# Autodesk Inventor assembly: 42146-28
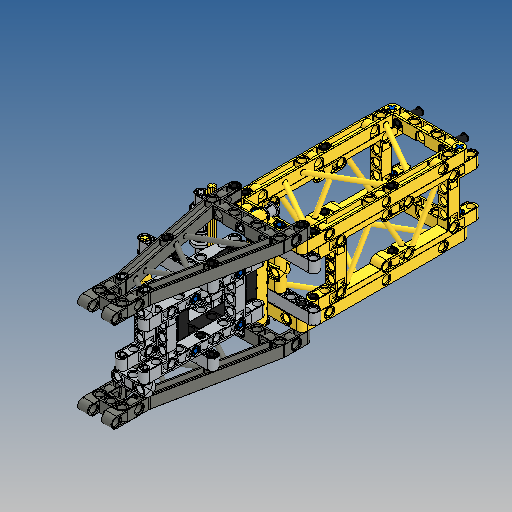
[picture p0: Inventor's stored thumbnail of the model, 512x512]
Saved by Autodesk Inventor 2025 (Build 290162010, 162A)
## iProperties
Created: 2024-12-04
Part Number: 42146-28
Material: Generisch
Document SubType Name: Assembly
Designer: hp.muther
Author: hp.muther
## Documents named in this file (22)
- D:\Inventor\Projekte\Muther\LEGO Technic\LEGO Technik - Raupenkran LR 13000 (42146)\42146-28.iam
- D:\Inventor\Projekte\Muther\LEGO Technic\LEGO Pieces\Rahmen, T-Stücke\79766-Yellow.ipt
- D:\Inventor\Projekte\Muther\LEGO Technic\LEGO Pieces\Pin's\2780-Black.ipt
- D:\Inventor\Projekte\Muther\LEGO Technic\LEGO Pieces\Pin's\43093-Blue.ipt
- D:\Inventor\Projekte\Muther\LEGO Technic\LEGO Pieces\Rahmen, T-Stücke\79767-Yellow.ipt
- D:\Inventor\Projekte\Muther\LEGO Technic\LEGO Pieces\Verbindungselemente\39793-Yellow.ipt
- D:\Inventor\Projekte\Muther\LEGO Technic\LEGO Pieces\Pin's\6558-Blue.ipt
- D:\Inventor\Projekte\Muther\LEGO Technic\LEGO Pieces\Lochbalken\32525-LtBluishGray.ipt
- D:\Inventor\Projekte\Muther\LEGO Technic\LEGO Pieces\Räder, Raupe\42610-LtBluishGray.ipt
- D:\Inventor\Projekte\Muther\LEGO Technic\LEGO Pieces\Rund\3713-LtBluishGray.ipt
- D:\Inventor\Projekte\Muther\LEGO Technic\LEGO Pieces\Rund\4265c-Yellow.ipt
- D:\Inventor\Projekte\Muther\LEGO Technic\LEGO Pieces\Achsen\32073-LtBluishGray.ipt
- D:\Inventor\Projekte\Muther\LEGO Technic\LEGO Pieces\Achsen\44294-Yellow.ipt
- D:\Inventor\Projekte\Muther\LEGO Technic\LEGO Pieces\Lochbalken\40490-Yellow.ipt
- D:\Inventor\Projekte\Muther\LEGO Technic\LEGO Pieces\Rahmen, T-Stücke\64178-LtBluishGray.ipt
- D:\Inventor\Projekte\Muther\LEGO Technic\LEGO Pieces\Rahmen, T-Stücke\64179-Black.ipt
- D:\Inventor\Projekte\Muther\LEGO Technic\LEGO Pieces\Verbindungselemente\48989-LtBluishGray.ipt
- D:\Inventor\Projekte\Muther\LEGO Technic\LEGO Pieces\Lochbalken\32524-LtBluishGray.ipt
- D:\Inventor\Projekte\Muther\LEGO Technic\LEGO Pieces\Rund\62462-Yellow.ipt
- D:\Inventor\Projekte\Muther\LEGO Technic\LEGO Pieces\Rahmen, T-Stücke\79768-DkBluishGray.ipt
- D:\Inventor\Projekte\Muther\LEGO Technic\LEGO Pieces\Pin's\18651-Black.ipt
- D:\Inventor\Projekte\Muther\LEGO Technic\LEGO Pieces\Pin's\32054-LtBluishGray.ipt
## Components (72 placed, 21 different names)
1. 79766-Yellow:1 — Einfügen:71, Einfügen:70, Einfügen:24, Einfügen:25, Einfügen:27, Einfügen:28, Einfügen:30, Einfügen:29, Einfügen:61, Einfügen:62, Einfügen:31, Einfügen:26, Einfügen:64
2. 2780-Black:1 — Einfügen:4
3. 2780-Black:2 — Einfügen:3
4. 2780-Black:3 — Einfügen:5
5. 2780-Black:4 — Einfügen:6
6. 2780-Black:5 — Einfügen:7
7. 43093-Blue:1 — Einfügen:2, Passend:2
8. 43093-Blue:2 — Einfügen:1, Passend:1
9. 79767-Yellow:1 — Einfügen:9, Passend:1
10. 79767-Yellow:2 — Einfügen:8, Passend:2, Einfügen:31, Passend:8
11. 39793-Yellow:1 — Einfügen:10, Einfügen:11, Einfügen:12, Einfügen:13, Einfügen:18, Einfügen:19
12. 6558-Blue:1 — Einfügen:10, Passend:7
13. 6558-Blue:2 — Einfügen:13
14. 6558-Blue:3 — Einfügen:11, Passend:3
15. 6558-Blue:4 — Einfügen:12
16. 32525-LtBluishGray:1 — Einfügen:19, Passend:4
17. 32525-LtBluishGray:2 — Einfügen:17, Einfügen:18, Passend:3, Einfügen:22, Einfügen:23
18. 42610-LtBluishGray:1 — Einfügen:16
19. 42610-LtBluishGray:2 — Einfügen:15, Einfügen:17
20. 3713-LtBluishGray:1 — Einfügen:14, Einfügen:15, Einfügen:16
21. 4265c-Yellow:1 — Einfügen:21, Passend:5
22. 4265c-Yellow:2 — Einfügen:20, Passend:6
23. 32073-LtBluishGray:1 — Einfügen:14, Passend:4
24. 44294-Yellow:1 — Einfügen:20, Einfügen:21, Passend:5, Passend:6, Einfügen:22
25. 79766-Yellow:2 — Einfügen:1, Einfügen:2, Einfügen:4, Einfügen:5, Einfügen:3, Einfügen:6, Einfügen:7, Einfügen:60, Einfügen:63, Einfügen:68, Einfügen:69, Passend:7, Einfügen:9, Einfügen:23, Einfügen:34, Einfügen:65, Einfügen:8
26. 2780-Black:6 — Einfügen:27
27. 2780-Black:7 — Einfügen:26, Passend:9
28. 2780-Black:8 — Einfügen:28
29. 2780-Black:9 — Einfügen:29
30. 2780-Black:10 — Einfügen:30
31. 43093-Blue:3 — Einfügen:25
32. 43093-Blue:4 — Einfügen:24, Passend:8
33. 6558-Blue:5 — Einfügen:32, Passend:18
34. 6558-Blue:6 — Einfügen:33
35. 40490-Yellow:1 — Einfügen:32, Einfügen:33, Einfügen:34, Passend:9, Einfügen:59, Einfügen:66, Einfügen:67
36. 64178-LtBluishGray:1 — Einfügen:40, Passend:11, Passend:12, Passend:13, Einfügen:47, Einfügen:58
37. 64179-Black:1 — Einfügen:39, Passend:10, Einfügen:40, Einfügen:59, Passend:18
38. 6558-Blue:7 — Einfügen:35
39. 6558-Blue:8 — Einfügen:37, Passend:11
40. 6558-Blue:9 — Einfügen:38
41. 6558-Blue:10 — Einfügen:36, Passend:10
42. 64178-LtBluishGray:2 — Einfügen:35, Einfügen:36, Einfügen:37, Einfügen:38, Einfügen:39, Einfügen:41, Einfügen:42, Passend:14, Passend:17
43. 48989-LtBluishGray:1 — Einfügen:42, Passend:13
44. 48989-LtBluishGray:2 — Einfügen:41, Passend:12
45. 2780-Black:11 — Einfügen:46
46. 2780-Black:12 — Einfügen:45
47. 2780-Black:13 — Einfügen:44
48. 2780-Black:14 — Einfügen:43, Passend:14
49. 32524-LtBluishGray:1 — Einfügen:43, Einfügen:44, Einfügen:45, Einfügen:46, Einfügen:47, Einfügen:53
50. 4265c-Yellow:3 — Einfügen:49
51. 4265c-Yellow:4 — Einfügen:48, Einfügen:50, Einfügen:53
52. 44294-Yellow:2 — Einfügen:48, Einfügen:52
53. 3713-LtBluishGray:2 — Einfügen:51, Einfügen:52
54. 42610-LtBluishGray:3 — Einfügen:50, Einfügen:49
55. 62462-Yellow:1 — Einfügen:51
56. 2780-Black:15
57. 2780-Black:16 — Einfügen:56
58. 2780-Black:17
59. 2780-Black:18 — Passend:17
60. 32524-LtBluishGray:2 — Einfügen:56, Einfügen:58
61. 79768-DkBluishGray:1 — Einfügen:64, Passend:20
62. 79768-DkBluishGray:2 — Einfügen:65, Passend:19
63. 18651-Black:1 — Einfügen:61, Passend:20
64. 18651-Black:2 — Einfügen:60, Passend:19
65. 18651-Black:3 — Einfügen:62
66. 18651-Black:4 — Einfügen:63
67. 32054-LtBluishGray:1 — Einfügen:67
68. 32054-LtBluishGray:2 — Einfügen:66
69. 2780-Black:19 — Einfügen:68
70. 2780-Black:20 — Einfügen:69
71. 2780-Black:21 — Einfügen:70
72. 2780-Black:22 — Einfügen:71
## Relationships (91: Insert 71, Mate 20)
- Einfügen:1 [Insert]: 43093-Blue:2 ↔ 79766-Yellow:2
- Einfügen:2 [Insert]: 43093-Blue:1 ↔ 79766-Yellow:2
- Einfügen:3 [Insert]: 2780-Black:2 ↔ 79766-Yellow:2
- Einfügen:4 [Insert]: 2780-Black:1 ↔ 79766-Yellow:2
- Einfügen:5 [Insert]: 2780-Black:3 ↔ 79766-Yellow:2
- Einfügen:6 [Insert]: 2780-Black:4 ↔ 79766-Yellow:2
- Einfügen:7 [Insert]: 2780-Black:5 ↔ 79766-Yellow:2
- Einfügen:8 [Insert]: 79767-Yellow:2 ↔ 79766-Yellow:2
- Einfügen:9 [Insert]: 79767-Yellow:1 ↔ 79766-Yellow:2
- Passend:1 [Mate]: 43093-Blue:2 ↔ 79767-Yellow:1
- Passend:2 [Mate]: 43093-Blue:1 ↔ 79767-Yellow:2
- Einfügen:10 [Insert]: 39793-Yellow:1 ↔ 6558-Blue:1
- Einfügen:11 [Insert]: 39793-Yellow:1 ↔ 6558-Blue:3
- Einfügen:12 [Insert]: 39793-Yellow:1 ↔ 6558-Blue:4
- Einfügen:13 [Insert]: 39793-Yellow:1 ↔ 6558-Blue:2
- Einfügen:14 [Insert] (-24 mm): 3713-LtBluishGray:1 ↔ 32073-LtBluishGray:1
- Einfügen:15 [Insert]: 42610-LtBluishGray:2 ↔ 3713-LtBluishGray:1
- Einfügen:16 [Insert]: 42610-LtBluishGray:1 ↔ 3713-LtBluishGray:1
- Einfügen:17 [Insert]: 32525-LtBluishGray:2 ↔ 42610-LtBluishGray:2
- Einfügen:18 [Insert]: 39793-Yellow:1 ↔ 32525-LtBluishGray:2
- Passend:3 [Mate]: 6558-Blue:3 ↔ 32525-LtBluishGray:2
- Einfügen:19 [Insert]: 39793-Yellow:1 ↔ 32525-LtBluishGray:1
- Passend:4 [Mate]: 32525-LtBluishGray:1 ↔ 32073-LtBluishGray:1
- Einfügen:20 [Insert] (-8 mm): 4265c-Yellow:2 ↔ 44294-Yellow:1
- Einfügen:21 [Insert] (-8 mm): 4265c-Yellow:1 ↔ 44294-Yellow:1
- Passend:5 [Mate]: 4265c-Yellow:1 ↔ 44294-Yellow:1
- Passend:6 [Mate]: 4265c-Yellow:2 ↔ 44294-Yellow:1
- Einfügen:22 [Insert] (-48 mm): 32525-LtBluishGray:2 ↔ 44294-Yellow:1
- Einfügen:23 [Insert]: 32525-LtBluishGray:2 ↔ 79766-Yellow:2
- Passend:7 [Mate]: 6558-Blue:1 ↔ 79766-Yellow:2
- Einfügen:24 [Insert]: 79766-Yellow:1 ↔ 43093-Blue:4
- Einfügen:25 [Insert]: 79766-Yellow:1 ↔ 43093-Blue:3
- Einfügen:26 [Insert]: 79766-Yellow:1 ↔ 2780-Black:7
- Einfügen:27 [Insert]: 79766-Yellow:1 ↔ 2780-Black:6
- Einfügen:28 [Insert]: 79766-Yellow:1 ↔ 2780-Black:8
- Einfügen:29 [Insert]: 79766-Yellow:1 ↔ 2780-Black:9
- Einfügen:30 [Insert]: 79766-Yellow:1 ↔ 2780-Black:10
- Einfügen:31 [Insert]: 79766-Yellow:1 ↔ 79767-Yellow:2
- Passend:8 [Mate]: 79767-Yellow:2 ↔ 43093-Blue:4
- Einfügen:32 [Insert]: 6558-Blue:5 ↔ 40490-Yellow:1
- Einfügen:33 [Insert]: 6558-Blue:6 ↔ 40490-Yellow:1
- Einfügen:34 [Insert]: 79766-Yellow:2 ↔ 40490-Yellow:1
- Passend:9 [Mate]: 2780-Black:7 ↔ 40490-Yellow:1
- Einfügen:35 [Insert]: 6558-Blue:7 ↔ 64178-LtBluishGray:2
- Einfügen:36 [Insert]: 6558-Blue:10 ↔ 64178-LtBluishGray:2
- Einfügen:37 [Insert]: 6558-Blue:8 ↔ 64178-LtBluishGray:2
- Einfügen:38 [Insert]: 6558-Blue:9 ↔ 64178-LtBluishGray:2
- Einfügen:39 [Insert]: 64179-Black:1 ↔ 64178-LtBluishGray:2
- Passend:10 [Mate]: 64179-Black:1 ↔ 6558-Blue:10
- Einfügen:40 [Insert]: 64178-LtBluishGray:1 ↔ 64179-Black:1
- Passend:11 [Mate]: 64178-LtBluishGray:1 ↔ 6558-Blue:8
- Einfügen:41 [Insert]: 64178-LtBluishGray:2 ↔ 48989-LtBluishGray:2
- Einfügen:42 [Insert]: 64178-LtBluishGray:2 ↔ 48989-LtBluishGray:1
- Passend:12 [Mate]: 64178-LtBluishGray:1 ↔ 48989-LtBluishGray:2
- Passend:13 [Mate]: 64178-LtBluishGray:1 ↔ 48989-LtBluishGray:1
- Einfügen:43 [Insert]: 2780-Black:14 ↔ 32524-LtBluishGray:1
- Einfügen:44 [Insert]: 2780-Black:13 ↔ 32524-LtBluishGray:1
- Einfügen:45 [Insert]: 2780-Black:12 ↔ 32524-LtBluishGray:1
- Einfügen:46 [Insert]: 2780-Black:11 ↔ 32524-LtBluishGray:1
- Einfügen:47 [Insert]: 64178-LtBluishGray:1 ↔ 32524-LtBluishGray:1
- Passend:14 [Mate]: 64178-LtBluishGray:2 ↔ 2780-Black:14
- Einfügen:48 [Insert] (-12 mm): 4265c-Yellow:4 ↔ 44294-Yellow:2
- Einfügen:49 [Insert]: 4265c-Yellow:3 ↔ 42610-LtBluishGray:3
- [Mate]: 4265c-Yellow:3 ↔ 44294-Yellow:2
- [Mate]: 4265c-Yellow:4 ↔ 44294-Yellow:2
- Einfügen:50 [Insert]: 4265c-Yellow:4 ↔ 42610-LtBluishGray:3
- Einfügen:51 [Insert]: 3713-LtBluishGray:2 ↔ 62462-Yellow:1
- Einfügen:52 [Insert] (-16 mm): 44294-Yellow:2 ↔ 3713-LtBluishGray:2
- Einfügen:53 [Insert]: 32524-LtBluishGray:1 ↔ 4265c-Yellow:4
- [Insert]: 2780-Black:18 ↔ 32524-LtBluishGray:2
- [Insert]: 2780-Black:17 ↔ 32524-LtBluishGray:2
- Einfügen:56 [Insert]: 2780-Black:16 ↔ 32524-LtBluishGray:2
- [Insert]: 2780-Black:15 ↔ 32524-LtBluishGray:2
- Einfügen:58 [Insert]: 64178-LtBluishGray:1 ↔ 32524-LtBluishGray:2
- Passend:17 [Mate]: 64178-LtBluishGray:2 ↔ 2780-Black:18
- Einfügen:59 [Insert]: 40490-Yellow:1 ↔ 64179-Black:1
- Passend:18 [Mate]: 6558-Blue:5 ↔ 64179-Black:1
- Einfügen:60 [Insert]: 79766-Yellow:2 ↔ 18651-Black:2
- Einfügen:61 [Insert]: 79766-Yellow:1 ↔ 18651-Black:1
- Einfügen:62 [Insert]: 79766-Yellow:1 ↔ 18651-Black:3
- Einfügen:63 [Insert]: 79766-Yellow:2 ↔ 18651-Black:4
- Einfügen:64 [Insert]: 79766-Yellow:1 ↔ 79768-DkBluishGray:1
- Einfügen:65 [Insert]: 79766-Yellow:2 ↔ 79768-DkBluishGray:2
- Passend:19 [Mate]: 79768-DkBluishGray:2 ↔ 18651-Black:2
- Passend:20 [Mate]: 79768-DkBluishGray:1 ↔ 18651-Black:1
- Einfügen:66 [Insert]: 40490-Yellow:1 ↔ 32054-LtBluishGray:2
- Einfügen:67 [Insert]: 40490-Yellow:1 ↔ 32054-LtBluishGray:1
- Einfügen:68 [Insert]: 79766-Yellow:2 ↔ 2780-Black:19
- Einfügen:69 [Insert]: 79766-Yellow:2 ↔ 2780-Black:20
- Einfügen:70 [Insert]: 79766-Yellow:1 ↔ 2780-Black:21
- Einfügen:71 [Insert]: 79766-Yellow:1 ↔ 2780-Black:22
## Named parameters: d31_d0 = 0 mm, d32_d1 = 0 mm, d33_d2 = 0 mm, d34_d3 = 0 mm, d35_d4 = 0 mm, d36_d5 = 0 mm, d37_d6 = 0 mm, d63_d24 = -12 mm, d64_d25 = 0 mm, d65_d26 = 0 mm, d66_d27 = 0 mm, d71_d57 = 0 mm, d72_d58 = 0 mm, d73_d59 = 0 mm, d74_d60 = 0 mm
